# Autodesk Inventor assembly: solid fighting bot
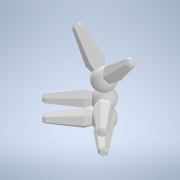
[picture p0: Inventor's stored thumbnail of the model, 180x180]
Saved by Autodesk Inventor 2022 (Build 260153000, 153)
## iProperties
Created: 2022-03-17
Part Number: solid fighting bot
Document SubType Name: Assembly
Designer: mogje
Author: mogje
## Documents named in this file (5)
- D:\Program Files (x86)\Autodesk Inventor\Projects\Microbots\solid fighting bot.iam
- D:\Program Files (x86)\Autodesk Inventor\Projects\Microbots\arms.ipt
- D:\Program Files (x86)\Autodesk Inventor\Projects\Microbots\solid bottom ball.ipt
- D:\Program Files (x86)\Autodesk Inventor\Projects\Microbots\solid mid ball.ipt
- D:\Program Files (x86)\Autodesk Inventor\Projects\Microbots\solid top ball.ipt
## Components (9 placed, 4 different names)
1. arms:1 — Mate:10, Mate:11
2. arms:2 — Mate:9, Mate:12
3. arms:3 — Mate:8, Mate:13
4. arms:4 — Mate:7, Mate:14
5. arms:5 — Mate:6, Mate:16
6. arms:6 — Mate:5, Mate:15
7. solid bottom ball:1 — Mate:3, Mate:4, Mate:5, Mate:6, Mate:15, Mate:16
8. solid mid ball:1 — Mate:1, Mate:2, Mate:3, Mate:4, Mate:7, Mate:8, Mate:13, Mate:14
9. solid top ball:1 — Mate:1, Mate:2, Mate:9, Mate:10, Mate:11, Mate:12
## Relationships (16: Mate 16)
- Mate:1: solid mid ball:1 ↔ solid top ball:1
- Mate:2: solid mid ball:1 ↔ solid top ball:1
- Mate:3: solid bottom ball:1 ↔ solid mid ball:1
- Mate:4: solid bottom ball:1 ↔ solid mid ball:1
- Mate:5: arms:6 ↔ solid bottom ball:1
- Mate:6: arms:5 ↔ solid bottom ball:1
- Mate:7: arms:4 ↔ solid mid ball:1
- Mate:8: arms:3 ↔ solid mid ball:1
- Mate:9: arms:2 ↔ solid top ball:1
- Mate:10: arms:1 ↔ solid top ball:1
- Mate:11: arms:1 ↔ solid top ball:1
- Mate:12: arms:2 ↔ solid top ball:1
- Mate:13: arms:3 ↔ solid mid ball:1
- Mate:14: arms:4 ↔ solid mid ball:1
- Mate:15: arms:6 ↔ solid bottom ball:1
- Mate:16: arms:5 ↔ solid bottom ball:1
